# Autodesk Inventor assembly: Full_Model
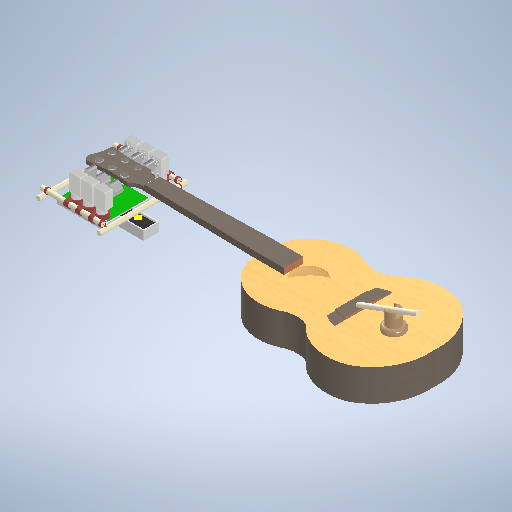
[picture p0: Inventor's stored thumbnail of the model, 512x512]
Saved by Autodesk Inventor 2025.2 (Build 292293000, 293)
## iProperties
Created: 2025-04-14
Part Number: Full_Model
Document SubType Name: Assembly
Designer: 3lin2
Author: 3lin2
## Documents named in this file (13)
- C:\Users\3lin2\OneDrive - University of Illinois - Urbana\Documents\UIUC\ECE 445\Automatic-Guitar-Tuner Github\3D_print\Full_Model.iam
- C:\Users\3lin2\OneDrive - University of Illinois - Urbana\Documents\UIUC\ECE 445\Automatic-Guitar-Tuner Github\3D_print\half_inch_dowel_5inch.ipt
- C:\Users\3lin2\OneDrive - University of Illinois - Urbana\Documents\UIUC\ECE 445\Automatic-Guitar-Tuner Github\3D_print\magnet_mount.ipt
- C:\Users\3lin2\OneDrive - University of Illinois - Urbana\Documents\UIUC\ECE 445\Automatic-Guitar-Tuner Github\3D_print\motor.ipt
- C:\Users\3lin2\OneDrive - University of Illinois - Urbana\Documents\UIUC\ECE 445\Automatic-Guitar-Tuner Github\3D_print\motor-tuningpeg.ipt
- C:\Users\3lin2\OneDrive - University of Illinois - Urbana\Documents\UIUC\ECE 445\Automatic-Guitar-Tuner Github\3D_print\Guitar.ipt
- C:\Users\3lin2\OneDrive - University of Illinois - Urbana\Documents\UIUC\ECE 445\Automatic-Guitar-Tuner Github\3D_print\tuningpeg.ipt
- C:\Users\3lin2\OneDrive - University of Illinois - Urbana\Documents\UIUC\ECE 445\Automatic-Guitar-Tuner Github\3D_print\motor-dowel.ipt
- C:\Users\3lin2\OneDrive - University of Illinois - Urbana\Documents\UIUC\ECE 445\Automatic-Guitar-Tuner Github\3D_print\PCB_mount.ipt
- C:\Users\3lin2\OneDrive - University of Illinois - Urbana\Documents\UIUC\ECE 445\Automatic-Guitar-Tuner Github\3D_print\dowel-dowel.ipt
- C:\Users\3lin2\OneDrive - University of Illinois - Urbana\Documents\UIUC\ECE 445\Automatic-Guitar-Tuner Github\3D_print\half_inch_dowel_10inch.ipt
- C:\Users\3lin2\OneDrive - University of Illinois - Urbana\Documents\UIUC\ECE 445\Automatic-Guitar-Tuner Github\3D_print\Battery.ipt
- C:\Users\3lin2\OneDrive - University of Illinois - Urbana\Documents\UIUC\ECE 445\Automatic-Guitar-Tuner Github\3D_print\PCB.ipt
## Components (38 placed, 12 different names)
1. half_inch_dowel_5inch:1 — Angle:1, Mate:2
2. magnet_mount:1 — Angle:1, Mate:1, Mate:2
3. motor:1 — Rotational:7, Flush:1, Mate:3, Mate:23, Mate:30, Flush:8, Flush:10
4. motor-tuningpeg:1 — Rotational:7
5. Guitar:1 — Mate:1, Rotational:1, Rotational:2, Rotational:3, Rotational:4, Rotational:5, Rotational:6, Flush:1, Mate:3, Flush:2, Mate:4, Mate:5, Flush:3, Mate:7, Mate:8, Flush:5, Flush:6, Mate:27, Mate:33, Mate:34
6. tuningpeg:1 — Rotational:1
7. tuningpeg:2 — Rotational:2
8. tuningpeg:3 — Rotational:3
9. tuningpeg:4 — Rotational:6
10. tuningpeg:5 — Rotational:4
11. tuningpeg:6 — Rotational:5
12. motor:2 — Flush:2, Mate:4, Mate:22, Flush:9, Flush:10, Mate:31, Mate:32
13. motor-tuningpeg:2
14. motor:3 — Mate:5, Flush:3, Flush:7, Mate:19, Mate:21, Flush:9, Mate:32
15. motor-tuningpeg:3
16. motor:4 — Mate:11, Mate:27, Flush:11
17. motor-tuningpeg:4
18. motor:5 — Mate:8, Flush:6, Mate:15
19. motor-tuningpeg:5
20. motor:6 — Mate:7, Flush:5, Mate:14, Flush:11
21. motor-tuningpeg:6
22. half_inch_dowel_5inch:2 — Flush:7, Mate:24, Mate:25, Mate:26, Flush:8, Mate:39, Mate:40, Mate:41, Mate:42
23. half_inch_dowel_5inch:3 — Mate:12, Mate:16, Mate:17, Mate:35, Mate:36, Mate:37, Mate:38
24. motor-dowel:1 — Mate:11, Mate:12
25. motor-dowel:2 — Mate:14, Mate:16
26. motor-dowel:3 — Mate:15, Mate:17
27. motor-dowel:4 — Mate:19, Mate:21, Mate:26
28. motor-dowel:5 — Mate:22, Mate:24, Mate:31
29. motor-dowel:6 — Mate:23, Mate:25, Mate:30
30. PCB_mount:1 — Mate:33, Mate:34, Mate:47, Mate:48, Mate:49, Mate:50, Mate:51, Mate:52
31. dowel-dowel:1 — Mate:35, Flush:12, Mate:38
32. dowel-dowel:2 — Mate:36, Flush:12, Mate:37
33. dowel-dowel:3 — Mate:39, Mate:42, Flush:13, Mate:46
34. dowel-dowel:4 — Mate:40, Mate:41, Flush:13
35. half_inch_dowel_10inch:1
36. Battery:1 — Mate:47, Mate:48, Mate:49
37. half_inch_dowel_10inch:2 — Mate:46
38. PCB:1 — Mate:50, Mate:51, Mate:52
## Relationships (66: Mate 41, RevoluteJoint 12, Flush 12, Angle 1)
- Angle:1 (-70 deg): half_inch_dowel_5inch:1 ↔ magnet_mount:1
- Mate:1: magnet_mount:1 ↔ Guitar:1
- Mate:2 (6.985 mm): half_inch_dowel_5inch:1 ↔ magnet_mount:1
- Rotational:1 [RevoluteJoint]: Guitar:1 ↔ tuningpeg:1
- Rotational:2 [RevoluteJoint]: Guitar:1 ↔ tuningpeg:2
- Rotational:3 [RevoluteJoint]: Guitar:1 ↔ tuningpeg:3
- Rotational:4 [RevoluteJoint]: Guitar:1 ↔ tuningpeg:5
- Rotational:5 [RevoluteJoint]: Guitar:1 ↔ tuningpeg:6
- Rotational:6 [RevoluteJoint]: Guitar:1 ↔ tuningpeg:4
- Rotational:7 [RevoluteJoint]: motor:1 ↔ motor-tuningpeg:1
- Flush:1 (-66.04 mm): motor:1 ↔ Guitar:1
- Mate:3 (50.8 mm): motor:1 ↔ Guitar:1
- [RevoluteJoint]: motor:2 ↔ motor-tuningpeg:2
- [RevoluteJoint]: motor:3 ↔ motor-tuningpeg:3
- Flush:2 (66.04 mm): Guitar:1 ↔ motor:2
- Mate:4 (50.8 mm): Guitar:1 ↔ motor:2
- Mate:5 (50.8 mm): Guitar:1 ↔ motor:3
- Flush:3 (66.04 mm): Guitar:1 ↔ motor:3
- [RevoluteJoint]: motor:4 ↔ motor-tuningpeg:4
- [RevoluteJoint]: motor:5 ↔ motor-tuningpeg:5
- [RevoluteJoint]: motor:6 ↔ motor-tuningpeg:6
- Mate:7 (50.8 mm): Guitar:1 ↔ motor:6
- Mate:8 (50.8 mm): Guitar:1 ↔ motor:5
- Flush:5 (66.04 mm): Guitar:1 ↔ motor:6
- Flush:6 (66.04 mm): Guitar:1 ↔ motor:5
- Flush:7 (-63.5 mm): motor:3 ↔ half_inch_dowel_5inch:2
- Mate:11: motor:4 ↔ motor-dowel:1
- Mate:12: half_inch_dowel_5inch:3 ↔ motor-dowel:1
- Mate:14: motor:6 ↔ motor-dowel:2
- Mate:15: motor:5 ↔ motor-dowel:3
- Mate:16: half_inch_dowel_5inch:3 ↔ motor-dowel:2
- Mate:17: half_inch_dowel_5inch:3 ↔ motor-dowel:3
- Mate:19: motor:3 ↔ motor-dowel:4
- Mate:21 (-7.62 mm): motor:3 ↔ motor-dowel:4
- Mate:22: motor:2 ↔ motor-dowel:5
- Mate:23: motor:1 ↔ motor-dowel:6
- Mate:24: half_inch_dowel_5inch:2 ↔ motor-dowel:5
- Mate:25: half_inch_dowel_5inch:2 ↔ motor-dowel:6
- Mate:26: half_inch_dowel_5inch:2 ↔ motor-dowel:4
- Mate:27 (50.8 mm): Guitar:1 ↔ motor:4
- Mate:30 (-7.62 mm): motor:1 ↔ motor-dowel:6
- Flush:8 (11.43 mm): motor:1 ↔ half_inch_dowel_5inch:2
- Flush:9: motor:2 ↔ motor:3
- Flush:10: motor:1 ↔ motor:2
- Mate:31 (-7.62 mm): motor:2 ↔ motor-dowel:5
- Mate:32 (3.302 mm): motor:2 ↔ motor:3
- Flush:11: motor:4 ↔ motor:6
- Mate:33 (95.25 mm): Guitar:1 ↔ PCB_mount:1
- Mate:34: Guitar:1 ↔ PCB_mount:1
- Mate:35: half_inch_dowel_5inch:3 ↔ dowel-dowel:1
- Mate:36: half_inch_dowel_5inch:3 ↔ dowel-dowel:2
- Flush:12: dowel-dowel:1 ↔ dowel-dowel:2
- Mate:37: half_inch_dowel_5inch:3 ↔ dowel-dowel:2
- Mate:38 (-12.7 mm): half_inch_dowel_5inch:3 ↔ dowel-dowel:1
- Mate:39: half_inch_dowel_5inch:2 ↔ dowel-dowel:3
- Mate:40: half_inch_dowel_5inch:2 ↔ dowel-dowel:4
- Mate:41: half_inch_dowel_5inch:2 ↔ dowel-dowel:4
- Mate:42 (-12.7 mm): half_inch_dowel_5inch:2 ↔ dowel-dowel:3
- Flush:13: dowel-dowel:3 ↔ dowel-dowel:4
- Mate:46: dowel-dowel:3 ↔ half_inch_dowel_10inch:2
- Mate:47 (1.27 mm): PCB_mount:1 ↔ Battery:1
- Mate:48: PCB_mount:1 ↔ Battery:1
- Mate:49 (1.27 mm): PCB_mount:1 ↔ Battery:1
- Mate:50: PCB_mount:1 ↔ PCB:1
- Mate:51: PCB_mount:1 ↔ PCB:1
- Mate:52: PCB_mount:1 ↔ PCB:1
## Named parameters: d28_d23 = 0 mm, d29_d24 = 121.376524 deg, d30_d23 = 0 mm, d31_d24 = 6.06693 deg, d36_d23 = 0 mm, d37_d24 = -19.491279 deg, d40_d23 = 0 mm, d41_d24 = -1.910793 deg, d42_d23 = 0 mm, d43_d24 = -1.910793 deg
